# Autodesk Inventor assembly: Y-Axis_new
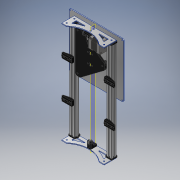
[picture p0: Inventor's stored thumbnail of the model, 180x180]
Saved by Autodesk Inventor 2020.3 (Build 243373000, 373)
## iProperties
Created: 2020-05-30
Part Number: Y-Axis_new
Document SubType Name: Assembly
Designer: rah75
Author: rah75
## Documents named in this file (17)
- C:\Users\rah75\Documents\GitHub\LETU-Maker\CAD\Autodesk Inventor\Base_3001-5999\Y-Axis\Assemblies\Y-Axis_new.iam
- C:\Users\rah75\Documents\GitHub\LETU-Maker\CAD\Autodesk Inventor\Base_3001-5999\Frame\Fabricated_Parts\Frame_Extrusion_20x20x400mm_LM3029.ipt
- C:\Users\rah75\Documents\GitHub\LETU-Maker\CAD\Autodesk Inventor\Base_3001-5999\Y-Axis\Fabricated_Parts\Y-Axis_Linear_Rod_1_4inx400mm_LM3038.ipt
- C:\Users\rah75\Documents\GitHub\LETU-Maker\CAD\Autodesk Inventor\Stock_Components_1001-2999\Motors\NEMA_17_LM1028.ipt
- C:\Users\rah75\Documents\GitHub\LETU-Maker\CAD\Autodesk Inventor\Stock_Components_1001-2999\Power_Transmission\Bearings\V-Groove_Bearing_5mm_LM1041.ipt
- C:\Users\rah75\Documents\GitHub\LETU-Maker\CAD\Autodesk Inventor\Base_3001-5999\Y-Carriage\Fabricated_Parts\Y-Carriage_Lower_Plate_LM3039.ipt
- C:\Users\rah75\Documents\GitHub\LETU-Maker\CAD\Autodesk Inventor\Stock_Components_1001-2999\Power_Transmission\GT2_pulley_LM1034.ipt
- C:\Users\rah75\Documents\GitHub\LETU-Maker\CAD\Autodesk Inventor\Base_3001-5999\Y-Axis\Printed_Parts\Y-Axis_Extrusion_Cap_LM3040.ipt
- C:\Users\rah75\Documents\GitHub\LETU-Maker\CAD\Autodesk Inventor\Base_3001-5999\Y-Axis\Printed_Parts\Y-Axis_Extursion_Mount_LM3041.ipt
- C:\Users\rah75\Documents\GitHub\LETU-Maker\CAD\Autodesk Inventor\Base_3001-5999\Y-Axis\Printed_Parts\Y-Axis_Motor_Mount_LM3042.ipt
- C:\Users\rah75\Documents\GitHub\LETU-Maker\CAD\Autodesk Inventor\Base_3001-5999\Y-Axis\Fabricated_Parts\Y-Axis_Cross_Bracket_LM3043.ipt
- C:\Users\rah75\Documents\GitHub\LETU-Maker\CAD\Autodesk Inventor\Base_3001-5999\Y-Carriage\Fabricated_Parts\Y-Carriage_Plate_LM3033_v2.ipt
- C:\Users\rah75\Documents\GitHub\LETU-Maker\CAD\Autodesk Inventor\Base_3001-5999\Y-Carriage\Printed_Parts\Y-Carraige_Spacer_LM3044.ipt
- C:\Users\rah75\Documents\GitHub\LETU-Maker\CAD\Autodesk Inventor\Base_3001-5999\Y-Axis\Printed_Parts\Y-Axis_Belt_Bearing_Mount_LM3045.ipt
- C:\Users\rah75\Documents\GitHub\LETU-Maker\CAD\Autodesk Inventor\Stock_Components_1001-2999\Power_Transmission\Bearings\625-ZZ_5x16mm_LM1030.ipt
- C:\Users\rah75\Documents\GitHub\LETU-Maker\CAD\Autodesk Inventor\Base_3001-5999\X-Carriage\Printed_Parts\X-Carriage_Belt_Clamp_LM3007.ipt
- C:\Users\rah75\Documents\GitHub\LETU-Maker\CAD\Autodesk Inventor\Stock_Components_1001-2999\Electrical\limit_switch_LM1025.ipt
## Components (30 placed, 16 different names)
1. Y-Axis_Cross_Bracket_LM3043:1 — Insert:3, Angle:1, Mate:19, Insert:12
2. Y-Axis_Cross_Bracket_LM3043:2 — Insert:1, Insert:2, Mate:17, Insert:18
3. Frame_Extrusion_20x20x400mm_LM3029:1 — Insert:2, Insert:3, Mate:2, Mate:4, Flush:1, Mate:10, Symmetry:1, Insert:8, Angle:3, Insert:9, Mate:15
4. Frame_Extrusion_20x20x400mm_LM3029:2 — Insert:1, Mate:1, Mate:3, Flush:2, Mate:11, Mate:12, Symmetry:1, Insert:7, Angle:2, Insert:10, Angle:4, Mate:14, Mate:16
5. Y-Axis_Linear_Rod_1_4inx400mm_LM3038:1 — Mate:2, Mate:5, Flush:1, Mate:6
6. Y-Axis_Linear_Rod_1_4inx400mm_LM3038:2 — Mate:1, Mate:3, Mate:4, Mate:5, Flush:2, Flush:6
7. NEMA_17_LM1028:1 — Insert:11, Insert:13
8. V-Groove_Bearing_5mm_LM1041:1 — Flush:5, Mate:7, Mate:8, Mate:9, Mate:11, Insert:4, Mate:20, Insert:16
9. V-Groove_Bearing_5mm_LM1041:2 — Flush:4, Mate:7, Mate:9, Mate:10, Insert:14, Insert:17
10. V-Groove_Bearing_5mm_LM1041:3 — Flush:4, Flush:5, Mate:6, Flush:6, Mate:8, Mate:12, Angle:1, Insert:5, Insert:15
11. Y-Carriage_Lower_Plate_LM3039:1 — Insert:4, Insert:5, Insert:20, Insert:21, Mate:21, Mate:22
12. GT2_pulley_LM1034:1 — Insert:11
13. Y-Axis_Extrusion_Cap_LM3040:1 — Insert:7, Angle:2
14. Y-Axis_Extrusion_Cap_LM3040:2 — Insert:8, Angle:3
15. Y-Axis_Extrusion_Cap_LM3040:3 — Insert:9
16. Y-Axis_Extrusion_Cap_LM3040:4 — Insert:10, Angle:4
17. Y-Axis_Extursion_Mount_LM3041:1 — Flush:7, Flush:8, Flush:9, Mate:14, Flush:12, Flush:14, Mate:17
18. Y-Axis_Extursion_Mount_LM3041:2 — Flush:10, Flush:11, Flush:13
19. Y-Axis_Extursion_Mount_LM3041:3 — Flush:9, Flush:10, Flush:11, Mate:15, Flush:12
20. Y-Axis_Extursion_Mount_LM3041:4 — Flush:7, Flush:8, Mate:16, Flush:13, Flush:14
21. Y-Axis_Motor_Mount_LM3042:1 — Mate:19, Insert:12, Insert:13
22. Y-Carriage_Plate_LM3033_v2:1 — Insert:14, Mate:20
23. Y-Carraige_Spacer_LM3044:1 — Insert:16
24. Y-Carraige_Spacer_LM3044:2 — Insert:17
25. Y-Carraige_Spacer_LM3044:3 — Insert:15
26. Y-Axis_Belt_Bearing_Mount_LM3045:2 — Insert:18, Insert:19
27. 625-ZZ_5x16mm_LM1030:1 — Insert:19
28. X-Carriage_Belt_Clamp_LM3007:1 — Insert:20, Mate:21
29. X-Carriage_Belt_Clamp_LM3007:2 — Insert:21, Mate:22
30. limit_switch_LM1025:1
## Relationships (58: Insert 20, Mate 20, Flush 13, Angle 4, Symmetry 1)
- Insert:1 (2 mm): Y-Axis_Cross_Bracket_LM3043:2 ↔ Frame_Extrusion_20x20x400mm_LM3029:2
- Insert:2 (2 mm): Y-Axis_Cross_Bracket_LM3043:2 ↔ Frame_Extrusion_20x20x400mm_LM3029:1
- Insert:3 (2 mm): Y-Axis_Cross_Bracket_LM3043:1 ↔ Frame_Extrusion_20x20x400mm_LM3029:1
- Mate:1 (11.0395 mm): Frame_Extrusion_20x20x400mm_LM3029:2 ↔ Y-Axis_Linear_Rod_1_4inx400mm_LM3038:2
- Mate:2 (11.0395 mm): Frame_Extrusion_20x20x400mm_LM3029:1 ↔ Y-Axis_Linear_Rod_1_4inx400mm_LM3038:1
- Mate:3: Frame_Extrusion_20x20x400mm_LM3029:2 ↔ Y-Axis_Linear_Rod_1_4inx400mm_LM3038:2
- Mate:4: Frame_Extrusion_20x20x400mm_LM3029:1 ↔ Y-Axis_Linear_Rod_1_4inx400mm_LM3038:2
- Mate:5: Y-Axis_Linear_Rod_1_4inx400mm_LM3038:1 ↔ Y-Axis_Linear_Rod_1_4inx400mm_LM3038:2
- Flush:1: Frame_Extrusion_20x20x400mm_LM3029:1 ↔ Y-Axis_Linear_Rod_1_4inx400mm_LM3038:1
- Flush:2: Frame_Extrusion_20x20x400mm_LM3029:2 ↔ Y-Axis_Linear_Rod_1_4inx400mm_LM3038:2
- Flush:4: V-Groove_Bearing_5mm_LM1041:2 ↔ V-Groove_Bearing_5mm_LM1041:3
- Flush:5: V-Groove_Bearing_5mm_LM1041:1 ↔ V-Groove_Bearing_5mm_LM1041:3
- Mate:6: Y-Axis_Linear_Rod_1_4inx400mm_LM3038:1 ↔ V-Groove_Bearing_5mm_LM1041:3
- Flush:6: Y-Axis_Linear_Rod_1_4inx400mm_LM3038:2 ↔ V-Groove_Bearing_5mm_LM1041:3
- Mate:7 (75 mm): V-Groove_Bearing_5mm_LM1041:1 ↔ V-Groove_Bearing_5mm_LM1041:2
- Mate:8 (150 mm): V-Groove_Bearing_5mm_LM1041:1 ↔ V-Groove_Bearing_5mm_LM1041:3
- Mate:9 (75 mm): V-Groove_Bearing_5mm_LM1041:1 ↔ V-Groove_Bearing_5mm_LM1041:2
- Mate:10 (15 mm): Frame_Extrusion_20x20x400mm_LM3029:1 ↔ V-Groove_Bearing_5mm_LM1041:2
- Mate:11 (15 mm): Frame_Extrusion_20x20x400mm_LM3029:2 ↔ V-Groove_Bearing_5mm_LM1041:1
- Mate:12 (15 mm): Frame_Extrusion_20x20x400mm_LM3029:2 ↔ V-Groove_Bearing_5mm_LM1041:3
- Angle:1 (0 deg): Y-Axis_Cross_Bracket_LM3043:1 ↔ V-Groove_Bearing_5mm_LM1041:3
- Insert:4: V-Groove_Bearing_5mm_LM1041:1 ↔ Y-Carriage_Lower_Plate_LM3039:1
- Insert:5: V-Groove_Bearing_5mm_LM1041:3 ↔ Y-Carriage_Lower_Plate_LM3039:1
- Symmetry:1: Frame_Extrusion_20x20x400mm_LM3029:1 ↔ Frame_Extrusion_20x20x400mm_LM3029:2
- Insert:7: Frame_Extrusion_20x20x400mm_LM3029:2 ↔ Y-Axis_Extrusion_Cap_LM3040:1
- Angle:2 (0 deg): Frame_Extrusion_20x20x400mm_LM3029:2 ↔ Y-Axis_Extrusion_Cap_LM3040:1
- Insert:8: Frame_Extrusion_20x20x400mm_LM3029:1 ↔ Y-Axis_Extrusion_Cap_LM3040:2
- Angle:3 (0 deg): Frame_Extrusion_20x20x400mm_LM3029:1 ↔ Y-Axis_Extrusion_Cap_LM3040:2
- Insert:9: Frame_Extrusion_20x20x400mm_LM3029:1 ↔ Y-Axis_Extrusion_Cap_LM3040:3
- Insert:10: Frame_Extrusion_20x20x400mm_LM3029:2 ↔ Y-Axis_Extrusion_Cap_LM3040:4
- Angle:4 (0 deg): Frame_Extrusion_20x20x400mm_LM3029:2 ↔ Y-Axis_Extrusion_Cap_LM3040:4
- Insert:11 (4.5 mm): NEMA_17_LM1028:1 ↔ GT2_pulley_LM1034:1
- Flush:7: Y-Axis_Extursion_Mount_LM3041:1 ↔ Y-Axis_Extursion_Mount_LM3041:4
- Flush:8: Y-Axis_Extursion_Mount_LM3041:1 ↔ Y-Axis_Extursion_Mount_LM3041:4
- Flush:9: Y-Axis_Extursion_Mount_LM3041:1 ↔ Y-Axis_Extursion_Mount_LM3041:3
- Flush:10: Y-Axis_Extursion_Mount_LM3041:2 ↔ Y-Axis_Extursion_Mount_LM3041:3
- Flush:11: Y-Axis_Extursion_Mount_LM3041:2 ↔ Y-Axis_Extursion_Mount_LM3041:3
- Mate:14: Frame_Extrusion_20x20x400mm_LM3029:2 ↔ Y-Axis_Extursion_Mount_LM3041:1
- Mate:15: Frame_Extrusion_20x20x400mm_LM3029:1 ↔ Y-Axis_Extursion_Mount_LM3041:3
- Mate:16: Frame_Extrusion_20x20x400mm_LM3029:2 ↔ Y-Axis_Extursion_Mount_LM3041:4
- Flush:12: Y-Axis_Extursion_Mount_LM3041:1 ↔ Y-Axis_Extursion_Mount_LM3041:3
- Flush:13: Y-Axis_Extursion_Mount_LM3041:2 ↔ Y-Axis_Extursion_Mount_LM3041:4
- Flush:14 (150 mm): Y-Axis_Extursion_Mount_LM3041:1 ↔ Y-Axis_Extursion_Mount_LM3041:4
- Mate:17 (115 mm): Y-Axis_Cross_Bracket_LM3043:2 ↔ Y-Axis_Extursion_Mount_LM3041:1
- Mate:19: Y-Axis_Cross_Bracket_LM3043:1 ↔ Y-Axis_Motor_Mount_LM3042:1
- Insert:12: Y-Axis_Cross_Bracket_LM3043:1 ↔ Y-Axis_Motor_Mount_LM3042:1
- Insert:13: NEMA_17_LM1028:1 ↔ Y-Axis_Motor_Mount_LM3042:1
- Insert:14 (8 mm): V-Groove_Bearing_5mm_LM1041:2 ↔ Y-Carriage_Plate_LM3033_v2:1
- Mate:20: V-Groove_Bearing_5mm_LM1041:1 ↔ Y-Carriage_Plate_LM3033_v2:1
- Insert:15: V-Groove_Bearing_5mm_LM1041:3 ↔ Y-Carraige_Spacer_LM3044:3
- Insert:16: V-Groove_Bearing_5mm_LM1041:1 ↔ Y-Carraige_Spacer_LM3044:1
- Insert:17: V-Groove_Bearing_5mm_LM1041:2 ↔ Y-Carraige_Spacer_LM3044:2
- Insert:18: Y-Axis_Cross_Bracket_LM3043:2 ↔ Y-Axis_Belt_Bearing_Mount_LM3045:2
- Insert:19 (1 mm): Y-Axis_Belt_Bearing_Mount_LM3045:2 ↔ 625-ZZ_5x16mm_LM1030:1
- Insert:20: Y-Carriage_Lower_Plate_LM3039:1 ↔ X-Carriage_Belt_Clamp_LM3007:1
- Insert:21: Y-Carriage_Lower_Plate_LM3039:1 ↔ X-Carriage_Belt_Clamp_LM3007:2
- Mate:21: Y-Carriage_Lower_Plate_LM3039:1 ↔ X-Carriage_Belt_Clamp_LM3007:1
- Mate:22: Y-Carriage_Lower_Plate_LM3039:1 ↔ X-Carriage_Belt_Clamp_LM3007:2
